# Autodesk Inventor assembly: Drive Train Actual
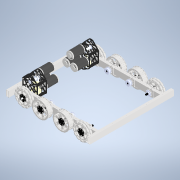
[picture p0: Inventor's stored thumbnail of the model, 180x180]
Saved by Autodesk Inventor 2020 (Build 240168000, 168)
## iProperties
Created: 2020-01-16
Part Number: Drive Train Actual
Document SubType Name: Assembly
Designer: aidan
Author: aidan
## Documents named in this file (8)
- C:\Users\aidan\Desktop\T3 Robotics\CAD\Drive Train Actual.iam
- C:\Users\aidan\Desktop\T3 Robotics\CAD\VerseFrame 28in Drive.ipt
- C:\Users\aidan\Desktop\T3 Robotics\CAD\VerseFrame 30in.ipt
- C:\Users\aidan\Desktop\T3 Robotics\CAD\VersaBlock Assembly.iam
- C:\Users\aidan\Desktop\T3 Robotics\CAD\WCP DS Gearbox.iam
- C:\Users\aidan\Desktop\T3 Robotics\CAD\Traction Wheel Assembly.iam
- C:\Users\aidan\Desktop\T3 Robotics\CAD\Omni Wheel Assembly.iam
- C:\Users\aidan\Desktop\T3 Robotics\CAD\Omni Wheel No Shaft.iam
## Components (20 placed, 7 different names)
1. VerseFrame 30in:1 — Mate:1, Flush:11, Flush:12
2. VerseFrame 30in:2 — Flush:13, Flush:14, Mate:2, Flush:15, Mate:14, Mate:15, Mate:16
3. VersaBlock Assembly:1 [sub-assembly] — Flush:8, Flush:18, Flush:24, Mate:21, Mate:24
4. VersaBlock Assembly:2 [sub-assembly] — Flush:7, Flush:8, Flush:18, Flush:19, Flush:23, Mate:20
5. VersaBlock Assembly:3 [sub-assembly] — Flush:7, Flush:19, Mate:5, Mate:6, Flush:22, Mate:19
6. VersaBlock Assembly:4 [sub-assembly] — Flush:10, Flush:16, Flush:21, Mate:3, Mate:16, Flush:24, Mate:18, Mate:23
7. VersaBlock Assembly:5 [sub-assembly] — Flush:9, Flush:10, Flush:17, Flush:20, Mate:13, Mate:14, Flush:22, Mate:22
8. VersaBlock Assembly:6 [sub-assembly] — Flush:9, Flush:16, Flush:17, Flush:20, Flush:21, Mate:4, Mate:15, Flush:23, Mate:17
9. VerseFrame 28in Drive:1 — Mate:1, Flush:11, Flush:12, Flush:13, Mate:5, Mate:6, Mate:7, Mate:8, Mate:9
10. VerseFrame 28in Drive:2 — Flush:14, Mate:2, Flush:15, Mate:3, Mate:4, Mate:10, Mate:11, Mate:12
11. WCP DS Gearbox:1 [sub-assembly] — Mate:7, Mate:8, Mate:9, Mate:26, Mate:28, Mate:30
12. WCP DS Gearbox:2 [sub-assembly] — Mate:10, Mate:11, Mate:12, Mate:25, Mate:27, Mate:29
13. Traction Wheel Assembly:1 [sub-assembly] — Mate:13, Mate:22, Flush:28, Rotation:1
14. Traction Wheel Assembly:2 [sub-assembly] — Mate:17, Flush:25, Flush:29, Rotation:1, Rotation:2
15. Traction Wheel Assembly:3 [sub-assembly] — Mate:19, Flush:26, Flush:28
16. Traction Wheel Assembly:4 [sub-assembly] — Mate:20, Flush:26, Flush:27, Flush:29
17. Omni Wheel Assembly:1 [sub-assembly] — Mate:18, Flush:25, Mate:23, Flush:30, Rotation:2
18. Omni Wheel Assembly:2 [sub-assembly] — Mate:21, Flush:27, Mate:24, Flush:30
19. Omni Wheel No Shaft:1 [sub-assembly] — Mate:25, Mate:27, Mate:29
20. Omni Wheel No Shaft:2 [sub-assembly] — Mate:26, Mate:28, Mate:30
## Relationships (56: Mate 30, Flush 24, RelateRotation 2)
- Flush:7: VersaBlock Assembly:2 ↔ VersaBlock Assembly:3
- Flush:8: VersaBlock Assembly:1 ↔ VersaBlock Assembly:2
- Flush:9: VersaBlock Assembly:5 ↔ VersaBlock Assembly:6
- Flush:10: VersaBlock Assembly:4 ↔ VersaBlock Assembly:5
- Mate:1: VerseFrame 30in:1 ↔ VerseFrame 28in Drive:1
- Flush:11 (76.2 mm): VerseFrame 30in:1 ↔ VerseFrame 28in Drive:1
- Flush:12: VerseFrame 30in:1 ↔ VerseFrame 28in Drive:1
- Flush:13: VerseFrame 30in:2 ↔ VerseFrame 28in Drive:1
- Flush:14: VerseFrame 30in:2 ↔ VerseFrame 28in Drive:2
- Mate:2: VerseFrame 30in:2 ↔ VerseFrame 28in Drive:2
- Flush:15 (-76.2 mm): VerseFrame 30in:2 ↔ VerseFrame 28in Drive:2
- Flush:16: VersaBlock Assembly:4 ↔ VersaBlock Assembly:6
- Flush:17: VersaBlock Assembly:5 ↔ VersaBlock Assembly:6
- Flush:18: VersaBlock Assembly:1 ↔ VersaBlock Assembly:2
- Flush:19: VersaBlock Assembly:2 ↔ VersaBlock Assembly:3
- Flush:20: VersaBlock Assembly:5 ↔ VersaBlock Assembly:6
- Flush:21: VersaBlock Assembly:4 ↔ VersaBlock Assembly:6
- Mate:3: VersaBlock Assembly:4 ↔ VerseFrame 28in Drive:2
- Mate:4: VersaBlock Assembly:6 ↔ VerseFrame 28in Drive:2
- Mate:5: VersaBlock Assembly:3 ↔ VerseFrame 28in Drive:1
- Mate:6: VersaBlock Assembly:3 ↔ VerseFrame 28in Drive:1
- Mate:7: VerseFrame 28in Drive:1 ↔ WCP DS Gearbox:1
- Mate:8: VerseFrame 28in Drive:1 ↔ WCP DS Gearbox:1
- Mate:9: VerseFrame 28in Drive:1 ↔ WCP DS Gearbox:1
- Mate:10: VerseFrame 28in Drive:2 ↔ WCP DS Gearbox:2
- Mate:11: VerseFrame 28in Drive:2 ↔ WCP DS Gearbox:2
- Mate:12: VerseFrame 28in Drive:2 ↔ WCP DS Gearbox:2
- Mate:13: VersaBlock Assembly:5 ↔ Traction Wheel Assembly:1
- Mate:14 (260.35 mm): VerseFrame 30in:2 ↔ VersaBlock Assembly:5
- Mate:15 (450.85 mm): VerseFrame 30in:2 ↔ VersaBlock Assembly:6
- Mate:16 (622.3 mm): VerseFrame 30in:2 ↔ VersaBlock Assembly:4
- Flush:22: VersaBlock Assembly:3 ↔ VersaBlock Assembly:5
- Flush:23: VersaBlock Assembly:2 ↔ VersaBlock Assembly:6
- Flush:24: VersaBlock Assembly:1 ↔ VersaBlock Assembly:4
- Mate:17: VersaBlock Assembly:6 ↔ Traction Wheel Assembly:2
- Mate:18: VersaBlock Assembly:4 ↔ Omni Wheel Assembly:1
- Mate:19: VersaBlock Assembly:3 ↔ Traction Wheel Assembly:3
- Mate:20: VersaBlock Assembly:2 ↔ Traction Wheel Assembly:4
- Mate:21: VersaBlock Assembly:1 ↔ Omni Wheel Assembly:2
- Mate:22: VersaBlock Assembly:5 ↔ Traction Wheel Assembly:1
- Flush:25: Traction Wheel Assembly:2 ↔ Omni Wheel Assembly:1
- Mate:23: VersaBlock Assembly:4 ↔ Omni Wheel Assembly:1
- Flush:26: Traction Wheel Assembly:3 ↔ Traction Wheel Assembly:4
- Flush:27: Traction Wheel Assembly:4 ↔ Omni Wheel Assembly:2
- Mate:24: VersaBlock Assembly:1 ↔ Omni Wheel Assembly:2
- Flush:28: Traction Wheel Assembly:1 ↔ Traction Wheel Assembly:3
- Flush:29: Traction Wheel Assembly:2 ↔ Traction Wheel Assembly:4
- Flush:30: Omni Wheel Assembly:1 ↔ Omni Wheel Assembly:2
- Rotation:1 [RelateRotation] (1 ul): Traction Wheel Assembly:1 ↔ Traction Wheel Assembly:2
- Rotation:2 [RelateRotation] (1 ul): Traction Wheel Assembly:2 ↔ Omni Wheel Assembly:1
- Mate:25: WCP DS Gearbox:2 ↔ Omni Wheel No Shaft:1
- Mate:26: WCP DS Gearbox:1 ↔ Omni Wheel No Shaft:2
- Mate:27: WCP DS Gearbox:2 ↔ Omni Wheel No Shaft:1
- Mate:28: WCP DS Gearbox:1 ↔ Omni Wheel No Shaft:2
- Mate:29: WCP DS Gearbox:2 ↔ Omni Wheel No Shaft:1
- Mate:30: WCP DS Gearbox:1 ↔ Omni Wheel No Shaft:2
